# Autodesk Inventor assembly: V3Puncher
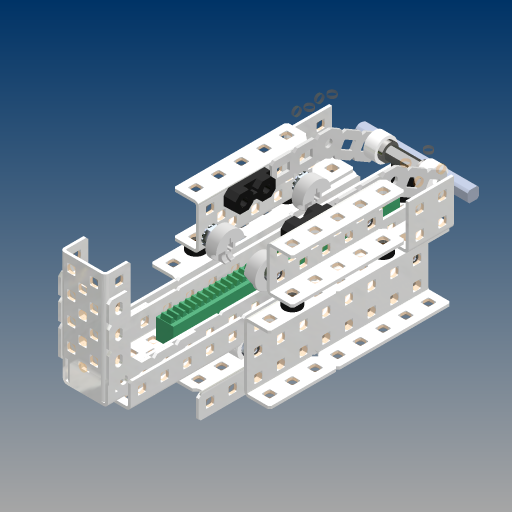
[picture p0: Inventor's stored thumbnail of the model, 512x512]
Saved by Autodesk Inventor 2023 (Build 270158000, 158)
## iProperties
Created: 2023-07-29
Part Number: V3Puncher
Document SubType Name: Assembly
Designer: eddie
Author: eddie
## Documents named in this file (28)
- C:\Users\eddie\Documents\81208X-Over-Under-CAD\V3\V3Puncher.iam
- C:\Users\eddie\Documents\81208X-Over-Under-CAD\VEX-CAD-Inventor-1.4.0\Structure\C Channel\Aluminum 1x3x1\Alu C 1x3x1x13.ipt
- C:\Users\eddie\Documents\81208X-Over-Under-CAD\VEX-CAD-Inventor-1.4.0\Structure\C Channel\Aluminum 1x3x1\Alu C 1x3x1x8.ipt
- C:\Users\eddie\Documents\81208X-Over-Under-CAD\VEX-CAD-Inventor-1.4.0\Structure\C Channel\Aluminum 1x3x1\Alu C 1x3x1x10.ipt
- C:\Users\eddie\Documents\81208X-Over-Under-CAD\VEX-CAD-Inventor-1.4.0\Motion\Spacers\Spacer Nylon .500 OD\NSpacer White .500 OD x .250.ipt
- C:\Users\eddie\Documents\81208X-Over-Under-CAD\VEX-CAD-Inventor-1.4.0\Motion\Spacers\Spacer Nylon .500 OD.ipt
- C:\Users\eddie\Documents\81208X-Over-Under-CAD\VEX-CAD-Inventor-1.4.0\Structure\Hardware\Nut Keps.ipt
- C:\Users\eddie\Documents\81208X-Over-Under-CAD\VEX-CAD-Inventor-1.4.0\Structure\Hardware\Nut Thin Nylock.ipt
- C:\Users\eddie\Documents\81208X-Over-Under-CAD\VEX-CAD-Inventor-1.4.0\Structure\C Channel\Aluminum 1x2x1\Alu C 1x2x1x15.ipt
- C:\Users\eddie\Documents\81208X-Over-Under-CAD\VEX-CAD-Inventor-1.4.0\Structure\Gussets\90 Plate Gusset.ipt
- C:\Users\eddie\Documents\81208X-Over-Under-CAD\VEX-CAD-Inventor-1.4.0\Motion\Spacers\Washer Steel\SWasher .375 OD x .031250.ipt
- C:\Users\eddie\Documents\81208X-Over-Under-CAD\VEX-CAD-Inventor-1.4.0\Motion\Spacers\Washer Steel.ipt
- C:\Users\eddie\Documents\81208X-Over-Under-CAD\VEX-CAD-Inventor-1.4.0\Motion\Spacers\Spacer Nylon .375 OD\NSpacer .375 OD x .125.ipt
- C:\Users\eddie\Documents\81208X-Over-Under-CAD\VEX-CAD-Inventor-1.4.0\Motion\Spacers\Spacer Nylon .375 OD.ipt
- C:\Users\eddie\Documents\81208X-Over-Under-CAD\VEX-CAD-Inventor-1.4.0\Structure\C Channel\Aluminum 1x2x1\Alu C 1x2x1x5.ipt
- C:\Users\eddie\Documents\81208X-Over-Under-CAD\Custom-parts\Bearing Flat with two holes.ipt
- C:\Users\eddie\Documents\81208X-Over-Under-CAD\VEX-CAD-Inventor-1.4.0\Structure\Gussets\30 Degree Flat Gusset.ipt
- C:\Users\eddie\Documents\81208X-Over-Under-CAD\Custom-parts\2x2 channel without 1 side.ipt
- C:\Users\eddie\Documents\81208X-Over-Under-CAD\VEX-CAD-Inventor-1.4.0\Motion\Advanced Gears\Rack Gear.ipt
- C:\Users\eddie\Documents\81208X-Over-Under-CAD\VEX-CAD-Inventor-1.4.0\Structure\Standoff\Standoff .75.ipt
- C:\Users\eddie\Documents\81208X-Over-Under-CAD\VEX-CAD-Inventor-1.4.0\Structure\Standoff.ipt
- C:\Users\eddie\Documents\81208X-Over-Under-CAD\VEX-CAD-Inventor-1.4.0\Structure\Gussets\C Channel Coupler.ipt
- C:\Users\eddie\Documents\81208X-Over-Under-CAD\VEX-CAD-Inventor-1.4.0\Structure\C Channel\Aluminum 1x2x1\Alu C 1x2x1x4.ipt
- C:\Users\eddie\Documents\81208X-Over-Under-CAD\VEX-CAD-Inventor-1.4.0\Motion\Spacers\Spacer Nylon .375 OD\NSpacer .375 OD x .250.ipt
- C:\Users\eddie\Documents\81208X-Over-Under-CAD\VEX-CAD-Inventor-1.4.0\Motion\Spacers\Spacer Nylon .375 OD\NSpacer .375 OD x .375.ipt
- C:\Users\eddie\Documents\81208X-Over-Under-CAD\VEX-CAD-Inventor-1.4.0\Motion\Shaft HS\Shaft HS\Shaft HS 2.5 in.ipt
- C:\Users\eddie\Documents\81208X-Over-Under-CAD\VEX-CAD-Inventor-1.4.0\Motion\Shaft HS\Shaft HS.ipt
- C:\Users\eddie\Downloads\Clamping Shaft Collar (276-3891).iam
## Components (65 placed, 22 different names)
1. Alu C 1x3x1x13:1 — Insert:1, Insert:2, Insert:16
2. Alu C 1x3x1x8:1 — Insert:1, Insert:3, Insert:4, Insert:10, Insert:19, Insert:21, Insert:38
3. Alu C 1x3x1x8:2 — Insert:2, Insert:6, Insert:12, Insert:20, Insert:22, Insert:37
4. Alu C 1x3x1x10:1 — Insert:3
5. NSpacer White .500 OD x .250:1 — Insert:5, Insert:9
6. NSpacer White .500 OD x .250:2 — Insert:7, Insert:8
7. Nut Keps:1 — Insert:4, Insert:5
8. Nut Keps:2 — Insert:6, Insert:7
9. Nut Thin Nylock:1 — Insert:9
10. Nut Thin Nylock:2 — Insert:8
11. NSpacer White .500 OD x .250:3 — Insert:11, Insert:15
12. NSpacer White .500 OD x .250:4 — Insert:13, Insert:14
13. Nut Keps:3 — Insert:10, Insert:11
14. Nut Keps:4 — Insert:12, Insert:13
15. Nut Thin Nylock:3 — Insert:15
16. Nut Thin Nylock:4 — Insert:14
17. Alu C 1x2x1x15:1 — Insert:16, Insert:17, Insert:18, Insert:39, Insert:40, Insert:50, Insert:52, Insert:53
18. 90 Plate Gusset:1 — Insert:18
19. 90 Plate Gusset:2 — Insert:17
20. SWasher .375 OD x .031250:1 — Insert:30, Insert:31
21. SWasher .375 OD x .031250:2 — Insert:29, Insert:30
22. SWasher .375 OD x .031250:3 — Insert:27, Insert:28
23. SWasher .375 OD x .031250:4 — Insert:28
24. SWasher .375 OD x .031250:5 — Insert:26
25. SWasher .375 OD x .031250:6 — Insert:25, Insert:26
26. SWasher .375 OD x .031250:7 — Insert:24, Insert:32
27. SWasher .375 OD x .031250:8 — Insert:23, Insert:24
28. NSpacer .375 OD x .125:1 — Insert:22, Insert:25
29. NSpacer .375 OD x .125:2 — Insert:21, Insert:27
30. NSpacer .375 OD x .125:3 — Insert:19, Insert:29
31. NSpacer .375 OD x .125:4 — Insert:20, Insert:23
32. Alu C 1x2x1x5:1 — Insert:31, Insert:33, Insert:35, Insert:58, Insert:59
33. Alu C 1x2x1x5:2 — Insert:32, Insert:34, Insert:36, Insert:56, Insert:57
34. Bearing Flat with two holes:1 — Insert:33
35. Bearing Flat with two holes:2 — Insert:34
36. 30 Degree Flat Gusset:1 — Insert:35, Insert:41
37. 30 Degree Flat Gusset:2 — Insert:36, Insert:42
38. 2x2 channel without 1 side:1 — Insert:37
39. 2x2 channel without 1 side:2 — Insert:38
40. Rack Gear:1 — Insert:39
41. Rack Gear:2 — Insert:40
42. NSpacer White .500 OD x .250:5 — Insert:42, Insert:46
43. NSpacer White .500 OD x .250:6 — Insert:41, Insert:43
44. SWasher .375 OD x .031250:9 — Insert:44, Insert:45
45. SWasher .375 OD x .031250:10 — Insert:43, Insert:44
46. SWasher .375 OD x .031250:11 — Insert:48, Insert:49
47. SWasher .375 OD x .031250:12 — Insert:47, Insert:48
48. SWasher .375 OD x .031250:13 — Insert:45
49. SWasher .375 OD x .031250:14 — Insert:46, Insert:47
50. Standoff .75:1 — Insert:49
51. C Channel Coupler:1 — Insert:50, Insert:51
52. Alu C 1x2x1x4:1 — Insert:51
53. NSpacer .375 OD x .250:5 — Insert:54
54. NSpacer .375 OD x .375:6 — Insert:52, Insert:54
55. NSpacer .375 OD x .250:7 — Insert:55, Mate:1
56. NSpacer .375 OD x .375:8 — Insert:53, Insert:55
57. Shaft HS 2.5 in:1 — Mate:1
58. Nut Keps:5 — Insert:56, Insert:61
59. Nut Keps:6 — Insert:57, Insert:63
60. Nut Keps:7 — Insert:58, Insert:60
61. Nut Keps:8 — Insert:59, Insert:62
62. Clamping Shaft Collar (276-3891):1 [sub-assembly] — Insert:60
63. Clamping Shaft Collar (276-3891):2 [sub-assembly] — Insert:62
64. Clamping Shaft Collar (276-3891):3 [sub-assembly] — Insert:63
65. Clamping Shaft Collar (276-3891):4 [sub-assembly] — Insert:61
## Relationships (64: Insert 63, Mate 1)
- Insert:1: Alu C 1x3x1x13:1 ↔ Alu C 1x3x1x8:1
- Insert:2: Alu C 1x3x1x13:1 ↔ Alu C 1x3x1x8:2
- Insert:3: Alu C 1x3x1x8:1 ↔ Alu C 1x3x1x10:1
- Insert:4: Alu C 1x3x1x8:1 ↔ Nut Keps:1
- Insert:5: NSpacer White .500 OD x .250:1 ↔ Nut Keps:1
- Insert:6: Alu C 1x3x1x8:2 ↔ Nut Keps:2
- Insert:7: NSpacer White .500 OD x .250:2 ↔ Nut Keps:2
- Insert:8: NSpacer White .500 OD x .250:2 ↔ Nut Thin Nylock:2
- Insert:9: NSpacer White .500 OD x .250:1 ↔ Nut Thin Nylock:1
- Insert:10: Alu C 1x3x1x8:1 ↔ Nut Keps:3
- Insert:11: NSpacer White .500 OD x .250:3 ↔ Nut Keps:3
- Insert:12: Alu C 1x3x1x8:2 ↔ Nut Keps:4
- Insert:13: NSpacer White .500 OD x .250:4 ↔ Nut Keps:4
- Insert:14: NSpacer White .500 OD x .250:4 ↔ Nut Thin Nylock:4
- Insert:15: NSpacer White .500 OD x .250:3 ↔ Nut Thin Nylock:3
- Insert:16: Alu C 1x3x1x13:1 ↔ Alu C 1x2x1x15:1
- Insert:17: Alu C 1x2x1x15:1 ↔ 90 Plate Gusset:2
- Insert:18: Alu C 1x2x1x15:1 ↔ 90 Plate Gusset:1
- Insert:19: Alu C 1x3x1x8:1 ↔ NSpacer .375 OD x .125:3
- Insert:20: Alu C 1x3x1x8:2 ↔ NSpacer .375 OD x .125:4
- Insert:21: Alu C 1x3x1x8:1 ↔ NSpacer .375 OD x .125:2
- Insert:22: Alu C 1x3x1x8:2 ↔ NSpacer .375 OD x .125:1
- Insert:23: SWasher .375 OD x .031250:8 ↔ NSpacer .375 OD x .125:4
- Insert:24: SWasher .375 OD x .031250:7 ↔ SWasher .375 OD x .031250:8
- Insert:25: SWasher .375 OD x .031250:6 ↔ NSpacer .375 OD x .125:1
- Insert:26: SWasher .375 OD x .031250:5 ↔ SWasher .375 OD x .031250:6
- Insert:27: SWasher .375 OD x .031250:3 ↔ NSpacer .375 OD x .125:2
- Insert:28: SWasher .375 OD x .031250:3 ↔ SWasher .375 OD x .031250:4
- Insert:29: SWasher .375 OD x .031250:2 ↔ NSpacer .375 OD x .125:3
- Insert:30: SWasher .375 OD x .031250:1 ↔ SWasher .375 OD x .031250:2
- Insert:31: SWasher .375 OD x .031250:1 ↔ Alu C 1x2x1x5:1
- Insert:32: SWasher .375 OD x .031250:7 ↔ Alu C 1x2x1x5:2
- Insert:33: Alu C 1x2x1x5:1 ↔ Bearing Flat with two holes:1
- Insert:34: Alu C 1x2x1x5:2 ↔ Bearing Flat with two holes:2
- Insert:35: Alu C 1x2x1x5:1 ↔ 30 Degree Flat Gusset:1
- Insert:36: Alu C 1x2x1x5:2 ↔ 30 Degree Flat Gusset:2
- Insert:37: Alu C 1x3x1x8:2 ↔ 2x2 channel without 1 side:1
- Insert:38: Alu C 1x3x1x8:1 ↔ 2x2 channel without 1 side:2
- Insert:39: Alu C 1x2x1x15:1 ↔ Rack Gear:1
- Insert:40: Alu C 1x2x1x15:1 ↔ Rack Gear:2
- Insert:41: 30 Degree Flat Gusset:1 ↔ NSpacer White .500 OD x .250:6
- Insert:42: 30 Degree Flat Gusset:2 ↔ NSpacer White .500 OD x .250:5
- Insert:43: NSpacer White .500 OD x .250:6 ↔ SWasher .375 OD x .031250:10
- Insert:44: SWasher .375 OD x .031250:9 ↔ SWasher .375 OD x .031250:10
- Insert:45: SWasher .375 OD x .031250:9 ↔ SWasher .375 OD x .031250:13
- Insert:46: NSpacer White .500 OD x .250:5 ↔ SWasher .375 OD x .031250:14
- Insert:47: SWasher .375 OD x .031250:12 ↔ SWasher .375 OD x .031250:14
- Insert:48: SWasher .375 OD x .031250:11 ↔ SWasher .375 OD x .031250:12
- Insert:49: SWasher .375 OD x .031250:11 ↔ Standoff .75:1
- Insert:50: Alu C 1x2x1x15:1 ↔ C Channel Coupler:1
- Insert:51: C Channel Coupler:1 ↔ Alu C 1x2x1x4:1
- Insert:52: Alu C 1x2x1x15:1 ↔ NSpacer .375 OD x .375:6
- Insert:53: Alu C 1x2x1x15:1 ↔ NSpacer .375 OD x .375:8
- Insert:54: NSpacer .375 OD x .250:5 ↔ NSpacer .375 OD x .375:6
- Insert:55: NSpacer .375 OD x .250:7 ↔ NSpacer .375 OD x .375:8
- Mate:1: NSpacer .375 OD x .250:7 ↔ Shaft HS 2.5 in:1
- Insert:56: Alu C 1x2x1x5:2 ↔ Nut Keps:5
- Insert:57: Alu C 1x2x1x5:2 ↔ Nut Keps:6
- Insert:58: Alu C 1x2x1x5:1 ↔ Nut Keps:7
- Insert:59: Alu C 1x2x1x5:1 ↔ Nut Keps:8
- Insert:60: Nut Keps:7 ↔ Clamping Shaft Collar (276-3891):1
- Insert:61: Nut Keps:5 ↔ Clamping Shaft Collar (276-3891):4
- Insert:62: Nut Keps:8 ↔ Clamping Shaft Collar (276-3891):2
- Insert:63: Nut Keps:6 ↔ Clamping Shaft Collar (276-3891):3
